# Autodesk Inventor assembly: ЛЦМК0000002.00.00.00.00.10
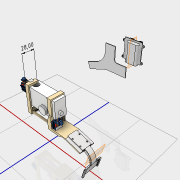
[picture p0: Inventor's stored thumbnail of the model, 180x180]
Saved by Autodesk Inventor 2021.2 (Build 252289000, 289)
## iProperties
Created: 2025-10-23
Part Number: ЛЦМК0000002.00.00.00.00.10
Document SubType Name: Assembly
Designer: Захаров
Author: Захаров
## Documents named in this file (12)
- C:\Users\User\Documents\CaseARHead1\ЛЦМК0000002.00.00.00.00.10.iam
- C:\Users\User\Documents\CaseARHead1\ЛЦМК0000002.00.00.00.00.05.ipt
- C:\Users\User\Documents\CaseARHead1\Сборка1.iam
- C:\Users\User\Documents\CaseARHead1\ЛЦМК000002.00.00.00.00.02.ipt
- C:\Users\User\Documents\CaseARHead1\ЛЦМК000002.00.00.00.00.07.ipt
- C:\Users\User\Documents\CaseARHead1\ЛЦМК000002.00.00.00.00.08.ipt
- C:\Users\User\Documents\CaseARHead1\ЛЦМК000002.00.00.00.00.09.ipt
- C:\Users\User\Documents\CaseARHead1\ЛЦМК000002.00.00.00.00.10.ipt
- C:\Users\User\Documents\CaseARHead1\ЛЦМК000002.00.00.00.00.06-04.ipt
- C:\Users\User\Documents\CaseARHead1\ЛЦМК000002.00.00.00.00.12.ipt
- C:\Users\User\Documents\CaseARHead1\ЛЦМК000002.00.00.00.00.13 OLED.ipt
- C:\Users\User\Documents\CaseARHead1\ЛЦМК000002.00.00.00.00.14 Фиксатор OLED.ipt
## Components (12 placed, 11 different names)
1. ЛЦМК0000002.00.00.00.00.05:1 — Заподлицо:8, Совмещение:2, Заподлицо:11
2. Сборка1:2 [sub-assembly] — Flush:7
3. ЛЦМК000002.00.00.00.00.06-04:1 — Совмещение:2, Совмещение:3, Заподлицо:11, Заподлицо:13, Заподлицо:14
4. ЛЦМК000002.00.00.00.00.02:1
5. ЛЦМК000002.00.00.00.00.07:1 — Flush:7
6. ЛЦМК000002.00.00.00.00.08:1 — Заподлицо:8, Заподлицо:12
7. ЛЦМК000002.00.00.00.00.09:1
8. ЛЦМК000002.00.00.00.00.10:1
9. Сборка1:3 [sub-assembly] — Совмещение:3
10. ЛЦМК000002.00.00.00.00.12:1 — Заподлицо:12
11. ЛЦМК000002.00.00.00.00.13 OLED:1 — Заподлицо:13
12. ЛЦМК000002.00.00.00.00.14 Фиксатор OLED:1 — Заподлицо:14
## Relationships (8: Flush 6, Mate 2)
- Flush:7: Сборка1:2 ↔ ЛЦМК000002.00.00.00.00.07:1
- Заподлицо:8 [Flush] (180 mm): ЛЦМК0000002.00.00.00.00.05:1 ↔ ЛЦМК000002.00.00.00.00.08:1
- Совмещение:2 [Mate]: ЛЦМК0000002.00.00.00.00.05:1 ↔ ЛЦМК000002.00.00.00.00.06-04:1
- Совмещение:3 [Mate]: ЛЦМК000002.00.00.00.00.06-04:1 ↔ Сборка1:3
- Заподлицо:11 [Flush] (7 mm): ЛЦМК0000002.00.00.00.00.05:1 ↔ ЛЦМК000002.00.00.00.00.06-04:1
- Заподлицо:12 [Flush]: ЛЦМК000002.00.00.00.00.08:1 ↔ ЛЦМК000002.00.00.00.00.12:1
- Заподлицо:13 [Flush]: ЛЦМК000002.00.00.00.00.06-04:1 ↔ ЛЦМК000002.00.00.00.00.13 OLED:1
- Заподлицо:14 [Flush]: ЛЦМК000002.00.00.00.00.06-04:1 ↔ ЛЦМК000002.00.00.00.00.14 Фиксатор OLED:1
